# Autodesk Inventor assembly: ForearmActuatorBody
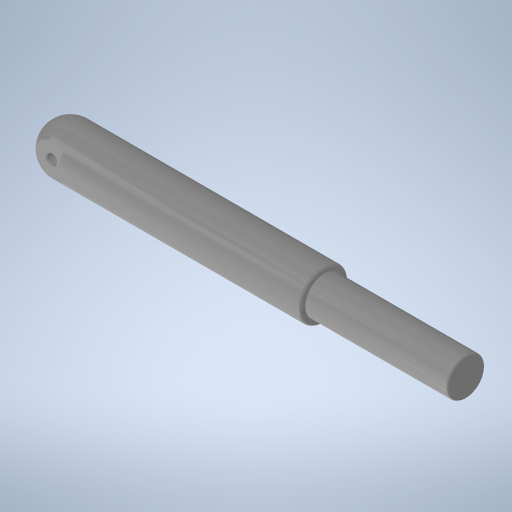
[picture p0: Inventor's stored thumbnail of the model, 512x512]
Saved by Autodesk Inventor 2023 (Build 270158000, 158)
## iProperties
Created: 2023-03-25
Part Number: ForearmActuatorBody
Document SubType Name: Assembly
Designer: Val
Mass: 762.816 g
Surface Area: 178.071 cm^2
Volume: 97.1741 cm^3
Density: 7.85 g/cm^3
Author: Val
## Documents named in this file (3)
- C:\Users\LattePanda\Desktop\str1ker\cad\external\ForearmActuator\ForearmActuatorBody.iam
- C:\Users\LattePanda\Desktop\str1ker\cad\external\ForearmActuator\ForearmActuatorBody.ipt
- C:\Users\LattePanda\Desktop\str1ker\cad\external\ForearmActuator\ForearmActuatorBodyBoundingBoxReal.ipt
## Components (2 placed, 2 different names)
1. ForearmActuatorBody:1 — Angle:2, Mate:1, Angle:3, Flush:1
2. ForearmActuatorBodyBoundingBoxReal:1 — Flush:1, Mate:2, Mate:3
## Relationships (6: Mate 3, Angle 2, Flush 1)
- Angle:2 (90 deg): ForearmActuatorBody:1
- Mate:1: ForearmActuatorBody:1
- Angle:3 (180 deg): ForearmActuatorBody:1
- Flush:1: ForearmActuatorBody:1 ↔ ForearmActuatorBodyBoundingBoxReal:1
- Mate:2: ForearmActuatorBodyBoundingBoxReal:1
- Mate:3: ForearmActuatorBodyBoundingBoxReal:1
